# Autodesk Inventor assembly: manifold assembly_MIR
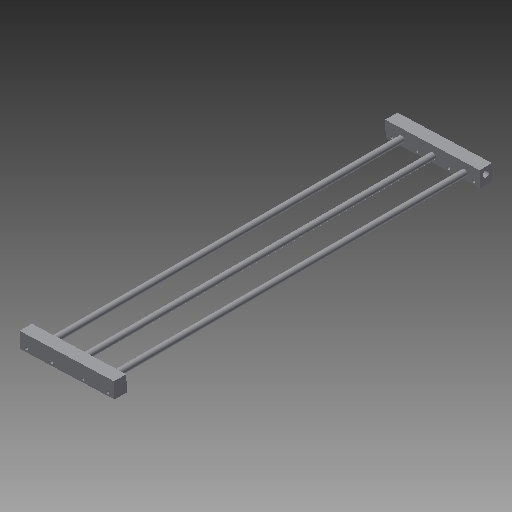
[picture p0: Inventor's stored thumbnail of the model, 512x512]
Saved by Autodesk Inventor 2018 (Build 220112000, 112)
## iProperties
Created: 2018-06-18
Part Number: manifold assembly_MIR
Document SubType Name: Assembly
Designer: John Viljoen
Author: John Viljoen
## Documents named in this file (3)
- C:\Users\John Viljoen\Documents\Inventor\computer project\manifold assembly_MIR.iam
- C:\Users\John Viljoen\Documents\Inventor\computer project\manifold mirror_MIR.ipt
- C:\Users\John Viljoen\Documents\Inventor\computer project\coverplate pipe_MIR.ipt
## Components (5 placed, 2 different names)
1. manifold mirror_MIR:1 — Mate:7, Mate:6, Mate:2, Mate:1, Mate:8
2. coverplate pipe_MIR:1 — Mate:7, Mate:6, Mate:5
3. coverplate pipe_MIR:2 — Mate:2, Mate:1, Mate:4, Mate:3
4. coverplate pipe_MIR:3 — Mate:8, Mate:9
5. manifold mirror_MIR:2 — Mate:9, Mate:5, Mate:4, Mate:3
## Relationships (9: Mate 9)
- Mate:7: manifold mirror_MIR:1 ↔ coverplate pipe_MIR:1
- Mate:6 (-5.2625 mm): manifold mirror_MIR:1 ↔ coverplate pipe_MIR:1
- Mate:2 (-5.2625 mm): manifold mirror_MIR:1 ↔ coverplate pipe_MIR:2
- Mate:1: manifold mirror_MIR:1 ↔ coverplate pipe_MIR:2
- Mate:8: manifold mirror_MIR:1 ↔ coverplate pipe_MIR:3
- Mate:9 (-5.2625 mm): coverplate pipe_MIR:3 ↔ manifold mirror_MIR:2
- Mate:5: coverplate pipe_MIR:1 ↔ manifold mirror_MIR:2
- Mate:4 (-5.2625 mm): coverplate pipe_MIR:2 ↔ manifold mirror_MIR:2
- Mate:3: coverplate pipe_MIR:2 ↔ manifold mirror_MIR:2
